# Autodesk Inventor assembly: SG90 - Micro Servo 9g - Tower Pro
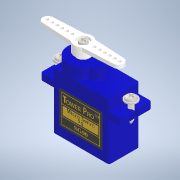
[picture p0: Inventor's stored thumbnail of the model, 180x180]
Saved by Autodesk Inventor 2022 (Build 260153000, 153)
## iProperties
Created: 2017-11-11
Part Number: SG90 - Micro Servo 9g - Tower Pro
Document SubType Name: Assembly
Designer: peter
Sending System: SolidWorks 2016
Last Author: mathe
Last Saved: 2017-11-11
Peso: 10.17
Projetista: Matheus A. Frasson
Data do Projeto: 00/00/0000
Data de Aprovação: 00/00/0000
Quantidade: 01
Revisão: Matheus A. Frasson
Aprovação: Matheus A. Frasson
Custo Total: 0.00
Author: peter
## Documents named in this file (5)
- C:\Users\peter\OneDrive\Desktop\sg90-micro-servo-9g-tower-pro-1.snapshot.3\Servo\SG90 - Micro Servo 9g - Tower Pro.iam
- C:\Users\peter\OneDrive\Desktop\sg90-micro-servo-9g-tower-pro-1.snapshot.3\SG90 - Micro Servo 9g - Tower Pro.1.ipt
- C:\Users\peter\OneDrive\Desktop\sg90-micro-servo-9g-tower-pro-1.snapshot.3\SG90 - Micro Servo 9g - Tower Pro.3.ipt
- C:\Users\peter\OneDrive\Desktop\sg90-micro-servo-9g-tower-pro-1.snapshot.3\SG90 - Micro Servo 9g - Tower Pro.5.ipt
- C:\Users\peter\OneDrive\Desktop\sg90-micro-servo-9g-tower-pro-1.snapshot.3\SG90 - Micro Servo 9g - Tower Pro.6.ipt
## Components (5 placed, 4 different names)
1. Tower Pro - Micro Servo 9g - SG90.1:1 — Rotational:1, Rotational:2
2. SG90 - Micro Servo 9g - Tower Pro.3:1
3. SG90 - Micro Servo 9g - Tower Pro.5:1 — Rotational:2
4. SG90 - Micro Servo 9g - Tower Pro.5:2 — Rotational:1
5. SG90 - Micro Servo 9g - Tower Pro.6:1
## Relationships (2: RevoluteJoint 2)
- Rotational:1 [RevoluteJoint] (2.5 mm): Tower Pro - Micro Servo 9g - SG90.1:1 ↔ SG90 - Micro Servo 9g - Tower Pro.5:2
- Rotational:2 [RevoluteJoint] (2.5 mm): Tower Pro - Micro Servo 9g - SG90.1:1 ↔ SG90 - Micro Servo 9g - Tower Pro.5:1
